# Autodesk Inventor assembly: MotorLeft
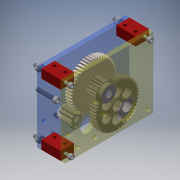
[picture p0: Inventor's stored thumbnail of the model, 180x180]
Saved by Autodesk Inventor 2019 (Build 230136000, 136)
## iProperties
Created: 2020-02-28
Part Number: MotorLeft
Document SubType Name: Assembly
Designer: james
Author: james
## Documents named in this file (22)
- F:\JimsRobot\FIRSTRobots\Design\TornadoPlatypus\MotorLeft.iam
- F:\JimsRobot\FIRSTRobots\Design\TornadoPlatypus\InsideMotorPlate.ipt
- F:\JimsRobot\FIRSTRobots\Design\Library\CTR\Falcon\217-6515 20191025.iam
- F:\JimsRobot\FIRSTRobots\Design\Library\AndyMark\FR6ZZ Bearing.ipt
- F:\JimsRobot\FIRSTRobots\Design\TornadoPlatypus\MotorSpacerBlock.ipt
- F:\JimsRobot\FIRSTRobots\Design\Library\AndyMark\Toughbox d07.ipt
- F:\JimsRobot\FIRSTRobots\Design\Library\AndyMark\6 HiGrip Asm Rev II.iam
- F:\JimsRobot\FIRSTRobots\Design\TornadoPlatypus\MotorSpacerBlock3.ipt
- F:\JimsRobot\FIRSTRobots\Design\Library\CTR\10T_20DP_FALCON.ipt
- F:\JimsRobot\FIRSTRobots\Design\Library\Fasteners\Size-10-32\HexCap-1.ipt
- F:\JimsRobot\FIRSTRobots\Design\Library\AndyMark\am-0149 50T 20dp 375hex REV2.ipt
- F:\JimsRobot\FIRSTRobots\Design\Library\AndyMark\am-0747 16t 20dp 375h with teeth.ipt
- F:\JimsRobot\FIRSTRobots\Design\Library\AndyMark\am-0184 48T 500in Hex Bore Gear REV2 (1).ipt
- F:\JimsRobot\FIRSTRobots\Design\TornadoPlatypus\OutsideMotorPlate.ipt
- F:\JimsRobot\FIRSTRobots\Design\Library\McMaster\Nuts\8-32 lock 90631A009_LOW-STRENGTH STEEL NYLON-INSERT LOCKNUT.ipt
- F:\JimsRobot\FIRSTRobots\Design\Library\McMaster\SocketScrews\8-32\2IN 91251A205_BLACK-OXIDE ALLOY STEEL SOCKET HEAD SCREW.ipt
- F:\JimsRobot\FIRSTRobots\Design\Library\McMaster\SocketScrews\8-32\1in 91251A199_BLACK-OXIDE ALLOY STEEL SOCKET HEAD CAP SCREW.ipt
- F:\JimsRobot\FIRSTRobots\Design\Library\AndyMark\500EX Hex Hub.ipt
- F:\JimsRobot\FIRSTRobots\Design\TornadoPlatypus\Shortend TB Output Shaft Hex L-Base 2.ipt
- F:\JimsRobot\FIRSTRobots\Design\Library\AndyMark\am-1526 500Hex HD Collar Clamp.iam
- F:\JimsRobot\FIRSTRobots\Design\Library\McMaster\6436K120_TWO-PIECE CLAMP-ON SHAFT COLLAR.ipt
- F:\JimsRobot\FIRSTRobots\Design\Library\AndyMark\FR8ZZ Hex Bearing.ipt
## Components (34 placed, 21 different names)
1. InsideMotorPlate:1 — Mate:1, Mate:2, Mate:3, Mate:5, Mate:6, Mate:8, Mate:9, Mate:10, Mate:11, Flush:1, Mate:13, Flush:3, Mate:14, Flush:4, Mate:42, Mate:44, Mate:45, Mate:46, Mate:50, Mate:59, Mate:60, Flush:11, Mate:84, Mate:89, Mate:92, Mate:93, Mate:98, Mate:111, Mate:112
2. 217-6515 20191025:1 [sub-assembly] — Mate:1, Mate:2, Mate:3, Mate:43
3. FR6ZZ Bearing:1 — Mate:5, Mate:6, Mate:15, Flush:5, Mate:48
4. MotorSpacerBlock:1 — Mate:9, Mate:13, Flush:3, Mate:26, Mate:28
5. MotorSpacerBlock:3 — Mate:10, Mate:11, Flush:1
6. MotorSpacerBlock:4 — Mate:8, Mate:14, Flush:4, Mate:27
7. Toughbox d07:1 — Mate:15, Flush:5, Mate:49, Mate:52, Mate:114
8. FR6ZZ Bearing:2 — Mate:111, Mate:112, Mate:115, Mate:116, Mate:118
9. OutsideMotorPlate:1 — Mate:26, Mate:27, Mate:28, Mate:29, Mate:30, Mate:85, Mate:86, Mate:96, Mate:97, Mate:100, Mate:101, Mate:113, Mate:121
10. 6 HiGrip Asm Rev II:1 [sub-assembly] — Mate:29, Mate:30, Mate:102, Mate:103, Mate:104
11. 10T_20DP_FALCON:1 — Mate:42, Mate:43
12. HexCap-1:1 — Mate:44, Mate:50
13. HexCap-1:2 — Mate:45, Mate:46
14. am-0149 50T 20dp 375hex REV2:1 — Mate:48, Mate:49, Mate:51, Mate:53
15. am-0747 16t 20dp 375h with teeth:1 — Mate:51, Mate:52
16. am-0184 48T 500in Hex Bore Gear REV2 (1):1 — Mate:53
17. MotorSpacerBlock3:3 — Mate:59, Mate:60, Flush:11, Mate:95
18. 8-32 lock 90631A009_LOW-STRENGTH STEEL NYLON-INSERT LOCKNUT:1 — Mate:84
19. 2IN 91251A205_BLACK-OXIDE ALLOY STEEL SOCKET HEAD SCREW:1 — Mate:85, Mate:86
20. 8-32 lock 90631A009_LOW-STRENGTH STEEL NYLON-INSERT LOCKNUT:2 — Mate:89
21. 1in 91251A199_BLACK-OXIDE ALLOY STEEL SOCKET HEAD CAP SCREW:1 — Mate:92, Mate:93, Mate:94
22. 8-32 lock 90631A009_LOW-STRENGTH STEEL NYLON-INSERT LOCKNUT:3 — Mate:94, Mate:95
23. 8-32 lock 90631A009_LOW-STRENGTH STEEL NYLON-INSERT LOCKNUT:6 — Mate:98, Mate:99
24. 2IN 91251A205_BLACK-OXIDE ALLOY STEEL SOCKET HEAD SCREW:2 — Mate:96, Mate:97, Mate:99
25. 2IN 91251A205_BLACK-OXIDE ALLOY STEEL SOCKET HEAD SCREW:3 — Mate:100, Mate:101
26. 500EX Hex Hub:1 — Mate:102, Mate:103, Mate:104, Mate:105, Mate:106, Mate:107, Mate:108, Mate:109, Mate:110, Mate:120
27. HexCap-1:3 — Mate:107, Mate:109
28. HexCap-1:4 — Mate:106, Mate:108
29. HexCap-1:5 — Mate:105, Mate:110
30. FR6ZZ Bearing:3 — Mate:113, Mate:114
31. Shortend TB Output Shaft Hex L-Base 2:1 — Mate:115, Mate:116, Mate:117, Mate:119
32. am-1526 500Hex HD Collar Clamp:1 [sub-assembly] — Mate:119, Mate:120
33. 6436K120_TWO-PIECE CLAMP-ON SHAFT COLLAR:1 — Mate:117, Mate:118, Mate:122
34. FR8ZZ Hex Bearing:1 — Mate:121, Mate:122
## Relationships (70: Mate 65, Flush 5)
- Mate:1: InsideMotorPlate:1 ↔ 217-6515 20191025:1
- Mate:2: InsideMotorPlate:1 ↔ 217-6515 20191025:1
- Mate:3: InsideMotorPlate:1 ↔ 217-6515 20191025:1
- Mate:5: InsideMotorPlate:1 ↔ FR6ZZ Bearing:1
- Mate:6: InsideMotorPlate:1 ↔ FR6ZZ Bearing:1
- Mate:8: InsideMotorPlate:1 ↔ MotorSpacerBlock:4
- Mate:9: InsideMotorPlate:1 ↔ MotorSpacerBlock:1
- Mate:10: InsideMotorPlate:1 ↔ MotorSpacerBlock:3
- Mate:11: InsideMotorPlate:1 ↔ MotorSpacerBlock:3
- Flush:1: InsideMotorPlate:1 ↔ MotorSpacerBlock:3
- Mate:13: InsideMotorPlate:1 ↔ MotorSpacerBlock:1
- Flush:3: InsideMotorPlate:1 ↔ MotorSpacerBlock:1
- Mate:14: InsideMotorPlate:1 ↔ MotorSpacerBlock:4
- Flush:4: InsideMotorPlate:1 ↔ MotorSpacerBlock:4
- Mate:15: FR6ZZ Bearing:1 ↔ Toughbox d07:1
- Flush:5: FR6ZZ Bearing:1 ↔ Toughbox d07:1
- Mate:26: MotorSpacerBlock:1 ↔ OutsideMotorPlate:1
- Mate:27: MotorSpacerBlock:4 ↔ OutsideMotorPlate:1
- Mate:28: MotorSpacerBlock:1 ↔ OutsideMotorPlate:1
- Mate:29: OutsideMotorPlate:1 ↔ 6 HiGrip Asm Rev II:1
- Mate:30: OutsideMotorPlate:1 ↔ 6 HiGrip Asm Rev II:1
- Mate:42: InsideMotorPlate:1 ↔ 10T_20DP_FALCON:1
- Mate:43: 217-6515 20191025:1 ↔ 10T_20DP_FALCON:1
- Mate:44: InsideMotorPlate:1 ↔ HexCap-1:1
- Mate:45: InsideMotorPlate:1 ↔ HexCap-1:2
- Mate:46: InsideMotorPlate:1 ↔ HexCap-1:2
- Mate:48: FR6ZZ Bearing:1 ↔ am-0149 50T 20dp 375hex REV2:1
- Mate:49: Toughbox d07:1 ↔ am-0149 50T 20dp 375hex REV2:1
- Mate:50: InsideMotorPlate:1 ↔ HexCap-1:1
- Mate:51: am-0149 50T 20dp 375hex REV2:1 ↔ am-0747 16t 20dp 375h with teeth:1
- Mate:52: Toughbox d07:1 ↔ am-0747 16t 20dp 375h with teeth:1
- Mate:53: am-0149 50T 20dp 375hex REV2:1 ↔ am-0184 48T 500in Hex Bore Gear REV2 (1):1
- Mate:59: InsideMotorPlate:1 ↔ MotorSpacerBlock3:3
- Mate:60: InsideMotorPlate:1 ↔ MotorSpacerBlock3:3
- Flush:11: InsideMotorPlate:1 ↔ MotorSpacerBlock3:3
- Mate:84: InsideMotorPlate:1 ↔ 8-32 lock 90631A009_LOW-STRENGTH STEEL NYLON-INSERT LOCKNUT:1
- Mate:85: OutsideMotorPlate:1 ↔ 2IN 91251A205_BLACK-OXIDE ALLOY STEEL SOCKET HEAD SCREW:1
- Mate:86: OutsideMotorPlate:1 ↔ 2IN 91251A205_BLACK-OXIDE ALLOY STEEL SOCKET HEAD SCREW:1
- Mate:89: InsideMotorPlate:1 ↔ 8-32 lock 90631A009_LOW-STRENGTH STEEL NYLON-INSERT LOCKNUT:2
- Mate:92: InsideMotorPlate:1 ↔ 1in 91251A199_BLACK-OXIDE ALLOY STEEL SOCKET HEAD CAP SCREW:1
- Mate:93: InsideMotorPlate:1 ↔ 1in 91251A199_BLACK-OXIDE ALLOY STEEL SOCKET HEAD CAP SCREW:1
- Mate:94: 1in 91251A199_BLACK-OXIDE ALLOY STEEL SOCKET HEAD CAP SCREW:1 ↔ 8-32 lock 90631A009_LOW-STRENGTH STEEL NYLON-INSERT LOCKNUT:3
- Mate:95: MotorSpacerBlock3:3 ↔ 8-32 lock 90631A009_LOW-STRENGTH STEEL NYLON-INSERT LOCKNUT:3
- Mate:96: OutsideMotorPlate:1 ↔ 2IN 91251A205_BLACK-OXIDE ALLOY STEEL SOCKET HEAD SCREW:2
- Mate:97: OutsideMotorPlate:1 ↔ 2IN 91251A205_BLACK-OXIDE ALLOY STEEL SOCKET HEAD SCREW:2
- Mate:98: InsideMotorPlate:1 ↔ 8-32 lock 90631A009_LOW-STRENGTH STEEL NYLON-INSERT LOCKNUT:6
- Mate:99: 8-32 lock 90631A009_LOW-STRENGTH STEEL NYLON-INSERT LOCKNUT:6 ↔ 2IN 91251A205_BLACK-OXIDE ALLOY STEEL SOCKET HEAD SCREW:2
- Mate:100: OutsideMotorPlate:1 ↔ 2IN 91251A205_BLACK-OXIDE ALLOY STEEL SOCKET HEAD SCREW:3
- Mate:101: OutsideMotorPlate:1 ↔ 2IN 91251A205_BLACK-OXIDE ALLOY STEEL SOCKET HEAD SCREW:3
- Mate:102: 6 HiGrip Asm Rev II:1 ↔ 500EX Hex Hub:1
- Mate:103: 6 HiGrip Asm Rev II:1 ↔ 500EX Hex Hub:1
- Mate:104: 6 HiGrip Asm Rev II:1 ↔ 500EX Hex Hub:1
- Mate:105: 500EX Hex Hub:1 ↔ HexCap-1:5
- Mate:106: 500EX Hex Hub:1 ↔ HexCap-1:4
- Mate:107: 500EX Hex Hub:1 ↔ HexCap-1:3
- Mate:108: 500EX Hex Hub:1 ↔ HexCap-1:4
- Mate:109: 500EX Hex Hub:1 ↔ HexCap-1:3
- Mate:110: 500EX Hex Hub:1 ↔ HexCap-1:5
- Mate:111: InsideMotorPlate:1 ↔ FR6ZZ Bearing:2
- Mate:112: InsideMotorPlate:1 ↔ FR6ZZ Bearing:2
- Mate:113: OutsideMotorPlate:1 ↔ FR6ZZ Bearing:3
- Mate:114: Toughbox d07:1 ↔ FR6ZZ Bearing:3
- Mate:115: FR6ZZ Bearing:2 ↔ Shortend TB Output Shaft Hex L-Base 2:1
- Mate:116: FR6ZZ Bearing:2 ↔ Shortend TB Output Shaft Hex L-Base 2:1
- Mate:117: Shortend TB Output Shaft Hex L-Base 2:1 ↔ 6436K120_TWO-PIECE CLAMP-ON SHAFT COLLAR:1
- Mate:118: FR6ZZ Bearing:2 ↔ 6436K120_TWO-PIECE CLAMP-ON SHAFT COLLAR:1
- Mate:119: Shortend TB Output Shaft Hex L-Base 2:1 ↔ am-1526 500Hex HD Collar Clamp:1
- Mate:120: 500EX Hex Hub:1 ↔ am-1526 500Hex HD Collar Clamp:1
- Mate:121: OutsideMotorPlate:1 ↔ FR8ZZ Hex Bearing:1
- Mate:122: 6436K120_TWO-PIECE CLAMP-ON SHAFT COLLAR:1 ↔ FR8ZZ Hex Bearing:1
